# Autodesk Inventor assembly: GGC
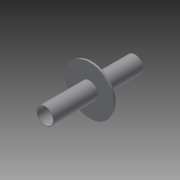
[picture p0: Inventor's stored thumbnail of the model, 180x180]
Saved by Autodesk Inventor 2015 (Build 190159000, 159)
## iProperties
Created: 2016-04-11
Part Number: GGC
Document SubType Name: Assembly
Designer: rubenjm
Author: rubenjm
## Documents named in this file (5)
- C:\Users\rubenjm\Documents\To Transfer\2k16 Spring\RME\GGC\GGC.iam
- C:\Users\rubenjm\Documents\To Transfer\2k16 Spring\RME\GGC\Inner Pole.ipt
- C:\Users\rubenjm\Documents\To Transfer\2k16 Spring\RME\GGC\Base Plate.ipt
- C:\Users\rubenjm\Documents\To Transfer\2k16 Spring\RME\GGC\Turntable_2.ipt
- C:\Users\rubenjm\Documents\To Transfer\2k16 Spring\RME\GGC\Top Plate.ipt
## Components (4 placed, 4 different names)
1. Inner Pole:1 — Flush:1, Mate:2, Mate:3, Cylindrical:1
2. Base Plate:1 — Flush:1, Mate:1, Mate:3, Mate:4
3. Turntable_2:1 — Mate:1, Mate:2, Mate:4, Mate:5
4. Top Plate:1 — Mate:5, Cylindrical:1
## Relationships (7: Mate 5, Flush 1, CylindricalJoint 1)
- Flush:1 (304.8 mm): Inner Pole:1 ↔ Base Plate:1
- Mate:1: Base Plate:1 ↔ Turntable_2:1
- Mate:2: Inner Pole:1 ↔ Turntable_2:1
- Mate:3: Inner Pole:1 ↔ Base Plate:1
- Mate:4: Base Plate:1 ↔ Turntable_2:1
- Mate:5: Turntable_2:1 ↔ Top Plate:1
- Cylindrical:1: Inner Pole:1 ↔ Top Plate:1
